# Autodesk Inventor assembly: Assembly1
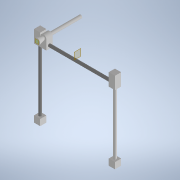
[picture p0: Inventor's stored thumbnail of the model, 180x180]
Saved by Autodesk Inventor 2021 (Build 250183000, 183)
## iProperties
Created: 2021-10-08
Part Number: Assembly1
Document SubType Name: Assembly
Designer: nikod
Author: nikod
## Documents named in this file (5)
- C:\Users\nikod\Documents\inzynierka\robo\Stare\1\Assembly1.iam
- C:\Users\nikod\Documents\inzynierka\robo\Stare\1\podstawa.ipt
- C:\Users\nikod\Documents\inzynierka\robo\Stare\1\srodek.ipt
- C:\Users\nikod\Documents\inzynierka\robo\Stare\1\klocek.ipt
- C:\Users\nikod\Documents\inzynierka\robo\Stare\1\ramie.ipt
## Components (4 placed, 4 different names)
1. podstawa:1 — Mate:1, Mate:2
2. srodek:1 — Mate:1, Mate:2, Mate:3, Flush:1
3. klocek:1 — Mate:3, Flush:1, Mate:4
4. ramie:1 — Mate:4
## Relationships (5: Mate 4, Flush 1)
- Mate:1: podstawa:1 ↔ srodek:1
- Mate:2: podstawa:1 ↔ srodek:1
- Mate:3: srodek:1 ↔ klocek:1
- Flush:1: srodek:1 ↔ klocek:1
- Mate:4: klocek:1 ↔ ramie:1
